# Autodesk Inventor assembly: Torretta
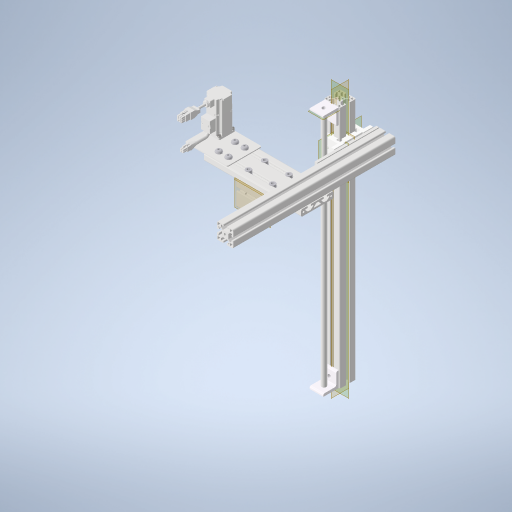
[picture p0: Inventor's stored thumbnail of the model, 512x512]
Saved by Autodesk Inventor 2023 (Build 270158000, 158)
## iProperties
Created: 2022-01-06
Part Number: Torretta
Document SubType Name: Assembly
Designer: matte
Author: matte
## Documents named in this file (10)
- C:\Users\matte\Documents\GitHub\MDM-CyberOrto-CAD\Torretta.iam
- C:\Users\matte\Documents\GitHub\MDM-CyberOrto-CAD\Carrello.iam
- C:\Users\matte\Documents\GitHub\MDM-CyberOrto-CAD\Parker components\08-Linear Application\01-Double Flange Slide Blocks\03-Metric Slide Blocks\30-4001.ipt
- C:\Users\matte\Documents\GitHub\MDM-CyberOrto-CAD\Parker components\03-Brackets_Gussets_Plates\07-Joining Plates\20-112.ipt
- C:\Users\matte\Documents\GitHub\MDM-CyberOrto-CAD\Pezzi singoli\Torretta\10-040.ipt
- C:\Users\matte\Documents\GitHub\MDM-CyberOrto-CAD\Parker components\02-Fasteners\10-Standard T-Nuts\20-058.ipt
- C:\Users\matte\Documents\GitHub\MDM-CyberOrto-CAD\Parker components\02-Fasteners\16-Screws\01-Metric Screws\01-Button Head\24-125-8.ipt
- C:\Users\matte\Documents\GitHub\MDM-CyberOrto-CAD\Parker components\02-Fasteners\10-Standard T-Nuts\20-050.ipt
- C:\Users\matte\Documents\GitHub\MDM-CyberOrto-CAD\Assiemi\Asta_verticale.iam
- C:\Users\matte\Documents\GitHub\MDM-CyberOrto-CAD\Rack_Pinion\Motor_assembly.iam
## Components (13 placed, 9 different names)
1. Carrello:1 [sub-assembly] — Coincidente:1, Coincidente:14, Allineato:8, Angolo:3, Tangente:1, Allineato:9, Coincidente:18, Coincidente:51, Allineato:12, Allineato:13
2. 10-040:1 — Coincidente:1, Allineato:6, Coincidente:5, Allineato:7, Angolo:1, Coincidente:7, Coincidente:12, Allineato:8, Coincidente:15, Angolo:4, Allineato:11
3. 20-050:1 — Coincidente:15, Angolo:4, Allineato:9, Coincidente:16, Coincidente:17, Allineato:11
4. 24-125-8:3 — Coincidente:16, Allineato:10, Coincidente:18
5. 24-125-8:4 — Coincidente:17, Allineato:10
6. Asta_verticale:1 [sub-assembly]
7. Motor_assembly:1 [sub-assembly] — Coincidente:51, Allineato:12, Allineato:13
8. 30-4001:1 — Coincidente:2, Coincidente:3, Coincidente:4, Coincidente:6, Coincidente:13
9. 20-112:1 — Coincidente:2, Coincidente:3, Coincidente:4, Allineato:6, Coincidente:5, Allineato:7, Coincidente:8, Coincidente:9, Coincidente:10, Coincidente:14
10. 20-058:1 — Angolo:1, Angolo:2, Coincidente:11, Coincidente:12
11. 24-125-8:1 — Coincidente:6, Coincidente:11, Coincidente:13
12. 20-058:2 — Angolo:2, Coincidente:7, Coincidente:8
13. 24-125-8:2 — Coincidente:9, Coincidente:10
## Relationships (34: Mate 21, Flush 8, Angle 4, Tangent 1)
- Coincidente:1 [Mate]: Carrello:1 ↔ 10-040:1
- Coincidente:2 [Mate]: 30-4001:1 ↔ 20-112:1
- Coincidente:3 [Mate]: 30-4001:1 ↔ 20-112:1
- Coincidente:4 [Mate]: 30-4001:1 ↔ 20-112:1
- Allineato:6 [Flush]: 10-040:1 ↔ 20-112:1
- Coincidente:5 [Mate]: 10-040:1 ↔ 20-112:1
- Allineato:7 [Flush]: 10-040:1 ↔ 20-112:1
- Coincidente:6 [Mate]: 30-4001:1 ↔ 24-125-8:1
- Angolo:1 [Angle] (180 deg): 10-040:1 ↔ 20-058:1
- Angolo:2 [Angle] (180 deg): 20-058:1 ↔ 20-058:2
- Coincidente:7 [Mate]: 10-040:1 ↔ 20-058:2
- Coincidente:8 [Mate]: 20-112:1 ↔ 20-058:2
- Coincidente:9 [Mate]: 20-112:1 ↔ 24-125-8:2
- Coincidente:10 [Mate]: 20-112:1 ↔ 24-125-8:2
- Coincidente:11 [Mate]: 20-058:1 ↔ 24-125-8:1
- Coincidente:12 [Mate]: 10-040:1 ↔ 20-058:1
- Coincidente:13 [Mate]: 30-4001:1 ↔ 24-125-8:1
- Coincidente:14 [Mate]: Carrello:1 ↔ 20-112:1
- Allineato:8 [Flush]: Carrello:1 ↔ 10-040:1
- Angolo:3 [Angle] (0 deg): Carrello:1
- Tangente:1: Carrello:1
- Coincidente:15 [Mate]: 10-040:1 ↔ 20-050:1
- Angolo:4 [Angle] (0 deg): 10-040:1 ↔ 20-050:1
- Allineato:9 [Flush] (-12.5 mm): Carrello:1 ↔ 20-050:1
- Coincidente:16 [Mate]: 20-050:1 ↔ 24-125-8:3
- Coincidente:17 [Mate]: 20-050:1 ↔ 24-125-8:4
- Allineato:10 [Flush]: 24-125-8:3 ↔ 24-125-8:4
- Coincidente:18 [Mate]: Carrello:1 ↔ 24-125-8:3
- Allineato:11 [Flush] (20 mm): 10-040:1 ↔ 20-050:1
- [Mate]: Asta_verticale:1 ↔ 30-4001:1
- [Mate]: Asta_verticale:1 ↔ 30-4001:1
- Coincidente:51 [Mate]: Carrello:1 ↔ Motor_assembly:1
- Allineato:12 [Flush]: Carrello:1 ↔ Motor_assembly:1
- Allineato:13 [Flush] (10 mm): Carrello:1 ↔ Motor_assembly:1
